# Autodesk Inventor assembly: PaddleCollection2.1.ipt
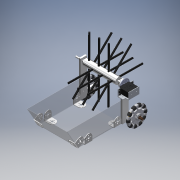
[picture p0: Inventor's stored thumbnail of the model, 180x180]
Saved by Autodesk Inventor 2019 (Build 230136000, 136)
## iProperties
Created: 2018-10-20
Part Number: PaddleCollection2.1.ipt
Document SubType Name: Assembly
Designer: User
Mass: 758.611 g
Surface Area: 3279.29 cm^2
Volume: 443.17 cm^3
Density: 1.71178 g/cm^3
Author: User
## Documents named in this file (20)
- C:\Robotics\CAD\2018-19_CAD\Collection\PaddleCollection2.1.ipt.iam
- C:\Robotics\CAD\2018-19_CAD\Collection\PaddleCollection2.1AxleSupport.ipt
- C:\Robotics\CAD\2018-19_CAD\Collection\PaddleCollection2.1Casing.ipt
- C:\Robotics\CAD\2018-19_CAD\Collection\PaddleCollectionFloor.ipt
- C:\Robotics\CAD\COTSParts\Tetrix\Tetrix Wheel 3 in omni.ipt
- C:\Robotics\CAD\COTSParts\Tetrix\Bronze bushing.ipt
- C:\Robotics\CAD\COTSParts\Tetrix\Tetrix shaft collar.ipt
- C:\Robotics\CAD\COTSParts\Tetrix\Tetrix Hub - axle.ipt
- C:\Robotics\CAD\COTSParts\Rev\REV-41-1097SmartServo.ipt
- C:\Robotics\CAD\COTSParts\Tetrix\39060_txm-standard servo bracket.ipt
- C:\Robotics\CAD\COTSParts\Tetrix\Tetrix bracket - angle.ipt
- C:\Robotics\CAD\2018-19_CAD\Collection\PaddleCollection2.1ServoSupport.ipt
- C:\Robotics\CAD\COTSParts\Bearings - AndyMark\Bearing 250 ID 500 OD flanged.ipt
- C:\Robotics\CAD\COTSParts\Actobotics\Collar.ipt
- C:\Robotics\CAD\COTSParts\Rev\REV-41-1363ServoHorn.ipt
- C:\Robotics\CAD\COTSParts\Actobotics\545 parts\545456PatternAdapter.77in.625in.ipt
- C:\Robotics\CAD\COTSParts\Actobotics\545 parts\545548SetScrewHub.77inPattern.ipt
- C:\Robotics\CAD\2018-19_CAD\Collection\SweeperAxle.ipt
- C:\Robotics\CAD\2018-19_CAD\Collection\SweeperSpoke.ipt
- C:\Robotics\CAD\2018-19_CAD\Collection\PaddleCollection2.1Backing.ipt
## Components (40 placed, 19 different names)
1. PaddleCollection2.1AxleSupport:1 — Mate:1, Mate:2, Flush:1, Insert:1, Insert:15, Mate:14
2. PaddleCollection2.1Casing:1 — Flush:3, Mate:5, Mate:6, Mate:1, Mate:13, Flush:6, Mate:40, Mate:41
3. PaddleCollection2.1Casing:2 — Mate:3, Mate:4, Flush:2, Flush:4, Mate:8, Flush:5, Mate:10, Mate:34, Mate:36, Mate:39
4. PaddleCollectionFloor:1 — Mate:2, Flush:1, Mate:3, Mate:4, Flush:2, Flush:3, Mate:5, Mate:6, Mate:9, Mate:12, Mate:35, Mate:37, Flush:7, Mate:43, Flush:10
5. Tetrix Wheel 3 in omni:1 — Insert:3, Insert:4
6. Bronze bushing:1 — Insert:1, Insert:2
7. Bronze bushing:2 — Insert:5
8. Tetrix shaft collar:1 — Insert:2, Insert:3
9. Tetrix Hub - axle:1 — Insert:4, Insert:5
10. REV-41-1097SmartServo:1 — Insert:6, Angle:1, Insert:17
11. 39060_txm-standard servo bracket:1 — Insert:6, Angle:1, Insert:7, Insert:8
12. Tetrix bracket - angle:1 — Insert:7, Insert:8, Insert:9, Angle:2
13. PaddleCollection2.1ServoSupport:1 — Flush:4, Mate:8, Flush:5, Insert:9, Angle:2, Insert:10, Mate:11
14. Bronze bushing:3 — Insert:14
15. Tetrix Wheel 3 in omni:2 — Insert:12, Insert:13
16. Tetrix shaft collar:2 — Insert:11, Insert:12
17. Tetrix Hub - axle:2 — Insert:13, Insert:14
18. Bronze bushing:4 — Insert:10, Insert:11
19. Bearing 250 ID 500 OD flanged:1 — Insert:15, Insert:16
20. Collar:1 — Insert:16
21. Tetrix bracket - angle:2 — Mate:9, Mate:10, Mate:11
22. Tetrix bracket - angle:3 — Mate:12, Mate:13, Mate:14
23. REV-41-1363ServoHorn:1 — Insert:17, Insert:18
24. 545456PatternAdapter.77in.625in:1 — Insert:18, Insert:19
25. 545548SetScrewHub.77inPattern:1 — Insert:19, Insert:20
26. SweeperAxle:1 — Mate:15, Mate:16, Mate:17, Mate:18, Mate:19, Mate:20, Mate:21, Mate:22, Mate:23, Mate:24, Mate:25, Mate:26, Mate:27, Mate:28, Mate:29, Mate:30, Mate:31, Mate:32, Mate:33, Insert:20
27. SweeperSpoke:1 — Mate:19, Mate:32
28. SweeperSpoke:2 — Mate:18, Mate:31
29. SweeperSpoke:3 — Mate:17, Mate:25
30. SweeperSpoke:4 — Mate:21, Mate:27, Mate:28
31. SweeperSpoke:5 — Mate:22, Mate:26
32. SweeperSpoke:6 — Mate:23, Mate:33
33. SweeperSpoke:7 — Mate:24, Mate:30
34. SweeperSpoke:8 — Mate:20, Mate:29
35. SweeperSpoke:9 — Mate:15, Mate:16
36. PaddleCollection2.1Backing:1 — Flush:6, Mate:34, Mate:35, Mate:38, Flush:8, Mate:42, Flush:9
37. Tetrix bracket - angle:4 — Mate:36, Mate:37, Flush:7
38. Tetrix bracket - angle:5 — Mate:38, Mate:39, Flush:8
39. Tetrix bracket - angle:6 — Mate:41, Mate:42, Flush:9
40. Tetrix bracket - angle:7 — Mate:40, Mate:43, Flush:10
## Relationships (74: Mate 42, Insert 20, Flush 10, Angle 2)
- Mate:1: PaddleCollection2.1AxleSupport:1 ↔ PaddleCollection2.1Casing:1
- Mate:2: PaddleCollection2.1AxleSupport:1 ↔ PaddleCollectionFloor:1
- Flush:1: PaddleCollection2.1AxleSupport:1 ↔ PaddleCollectionFloor:1
- Mate:3: PaddleCollection2.1Casing:2 ↔ PaddleCollectionFloor:1
- Mate:4: PaddleCollection2.1Casing:2 ↔ PaddleCollectionFloor:1
- Flush:2: PaddleCollection2.1Casing:2 ↔ PaddleCollectionFloor:1
- Flush:3: PaddleCollection2.1Casing:1 ↔ PaddleCollectionFloor:1
- Mate:5: PaddleCollection2.1Casing:1 ↔ PaddleCollectionFloor:1
- Mate:6: PaddleCollection2.1Casing:1 ↔ PaddleCollectionFloor:1
- Insert:1: PaddleCollection2.1AxleSupport:1 ↔ Bronze bushing:1
- Insert:2: Bronze bushing:1 ↔ Tetrix shaft collar:1
- Insert:3: Tetrix Wheel 3 in omni:1 ↔ Tetrix shaft collar:1
- Insert:4: Tetrix Wheel 3 in omni:1 ↔ Tetrix Hub - axle:1
- Insert:5: Bronze bushing:2 ↔ Tetrix Hub - axle:1
- Insert:6: REV-41-1097SmartServo:1 ↔ 39060_txm-standard servo bracket:1
- Angle:1 (0 deg): REV-41-1097SmartServo:1 ↔ 39060_txm-standard servo bracket:1
- Insert:7: 39060_txm-standard servo bracket:1 ↔ Tetrix bracket - angle:1
- Insert:8: 39060_txm-standard servo bracket:1 ↔ Tetrix bracket - angle:1
- Flush:4: PaddleCollection2.1Casing:2 ↔ PaddleCollection2.1ServoSupport:1
- Mate:8: PaddleCollection2.1Casing:2 ↔ PaddleCollection2.1ServoSupport:1
- Flush:5: PaddleCollection2.1Casing:2 ↔ PaddleCollection2.1ServoSupport:1
- Insert:9: Tetrix bracket - angle:1 ↔ PaddleCollection2.1ServoSupport:1
- Angle:2 (0 deg): Tetrix bracket - angle:1 ↔ PaddleCollection2.1ServoSupport:1
- Insert:10: PaddleCollection2.1ServoSupport:1 ↔ Bronze bushing:4
- Insert:11: Tetrix shaft collar:2 ↔ Bronze bushing:4
- Insert:12: Tetrix Wheel 3 in omni:2 ↔ Tetrix shaft collar:2
- Insert:13: Tetrix Wheel 3 in omni:2 ↔ Tetrix Hub - axle:2
- Insert:14: Bronze bushing:3 ↔ Tetrix Hub - axle:2
- Insert:15: PaddleCollection2.1AxleSupport:1 ↔ Bearing 250 ID 500 OD flanged:1
- Insert:16: Bearing 250 ID 500 OD flanged:1 ↔ Collar:1
- Mate:9: PaddleCollectionFloor:1 ↔ Tetrix bracket - angle:2
- Mate:10: PaddleCollection2.1Casing:2 ↔ Tetrix bracket - angle:2
- Mate:11: PaddleCollection2.1ServoSupport:1 ↔ Tetrix bracket - angle:2
- Mate:12: PaddleCollectionFloor:1 ↔ Tetrix bracket - angle:3
- Mate:13: PaddleCollection2.1Casing:1 ↔ Tetrix bracket - angle:3
- Mate:14: PaddleCollection2.1AxleSupport:1 ↔ Tetrix bracket - angle:3
- Insert:17: REV-41-1097SmartServo:1 ↔ REV-41-1363ServoHorn:1
- Insert:18: REV-41-1363ServoHorn:1 ↔ 545456PatternAdapter.77in.625in:1
- Insert:19: 545456PatternAdapter.77in.625in:1 ↔ 545548SetScrewHub.77inPattern:1
- Mate:15: SweeperAxle:1 ↔ SweeperSpoke:9
- Mate:16 (-106.3625 mm): SweeperAxle:1 ↔ SweeperSpoke:9
- Mate:17: SweeperAxle:1 ↔ SweeperSpoke:3
- Mate:18: SweeperAxle:1 ↔ SweeperSpoke:2
- Mate:19: SweeperAxle:1 ↔ SweeperSpoke:1
- Mate:20: SweeperAxle:1 ↔ SweeperSpoke:8
- Mate:21: SweeperAxle:1 ↔ SweeperSpoke:4
- Mate:22: SweeperAxle:1 ↔ SweeperSpoke:5
- Mate:23: SweeperAxle:1 ↔ SweeperSpoke:6
- Mate:24: SweeperAxle:1 ↔ SweeperSpoke:7
- Mate:25 (-106.3625 mm): SweeperAxle:1 ↔ SweeperSpoke:3
- Mate:26 (-106.3625 mm): SweeperAxle:1 ↔ SweeperSpoke:5
- Mate:27 (-106.3625 mm): SweeperAxle:1 ↔ SweeperSpoke:4
- Mate:28 (-106.3625 mm): SweeperAxle:1 ↔ SweeperSpoke:4
- Mate:29 (-106.3625 mm): SweeperAxle:1 ↔ SweeperSpoke:8
- Mate:30 (-106.3625 mm): SweeperAxle:1 ↔ SweeperSpoke:7
- Mate:31 (-106.3625 mm): SweeperAxle:1 ↔ SweeperSpoke:2
- Mate:32 (-106.3625 mm): SweeperAxle:1 ↔ SweeperSpoke:1
- Mate:33 (-106.3625 mm): SweeperAxle:1 ↔ SweeperSpoke:6
- Flush:6: PaddleCollection2.1Casing:1 ↔ PaddleCollection2.1Backing:1
- Mate:34: PaddleCollection2.1Casing:2 ↔ PaddleCollection2.1Backing:1
- Mate:35: PaddleCollectionFloor:1 ↔ PaddleCollection2.1Backing:1
- Mate:36: PaddleCollection2.1Casing:2 ↔ Tetrix bracket - angle:4
- Mate:37: PaddleCollectionFloor:1 ↔ Tetrix bracket - angle:4
- Flush:7 (-25.4 mm): PaddleCollectionFloor:1 ↔ Tetrix bracket - angle:4
- Mate:38: PaddleCollection2.1Backing:1 ↔ Tetrix bracket - angle:5
- Mate:39: PaddleCollection2.1Casing:2 ↔ Tetrix bracket - angle:5
- Flush:8: PaddleCollection2.1Backing:1 ↔ Tetrix bracket - angle:5
- Mate:40: PaddleCollection2.1Casing:1 ↔ Tetrix bracket - angle:7
- Mate:41: PaddleCollection2.1Casing:1 ↔ Tetrix bracket - angle:6
- Mate:42: PaddleCollection2.1Backing:1 ↔ Tetrix bracket - angle:6
- Flush:9: PaddleCollection2.1Backing:1 ↔ Tetrix bracket - angle:6
- Mate:43: PaddleCollectionFloor:1 ↔ Tetrix bracket - angle:7
- Flush:10 (25.4 mm): PaddleCollectionFloor:1 ↔ Tetrix bracket - angle:7
- Insert:20 (6.35 mm): 545548SetScrewHub.77inPattern:1 ↔ SweeperAxle:1
